# Autodesk Inventor assembly: Zahnriemen 16mm
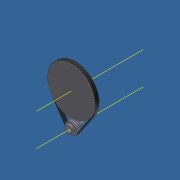
[picture p0: Inventor's stored thumbnail of the model, 180x180]
Saved by Autodesk Inventor 2016 (Build 200138000, 138)
## iProperties
Created: 2015-01-06
Document SubType Name: Assembly
Designer: 4ndreas
Mass: 1893.12 g
Surface Area: 594.287 cm^2
Volume: 258.329 cm^3
Density: 7.32831 g/cm^3
Part Number: Zahnriemen 16mm
ClientObjectVersion: 1
Author: 4ndreas
Title: 16mm Riemen
## Documents named in this file (4)
- C:\Users\4ndreas\Documents\Inventor\RobotARM v2\v2\BaseJoint\Konstruktions-Assistent\Übertragung des Zahnriemens1.iam
- C:\Users\4ndreas\Documents\Inventor\RobotARM v2\v2\BaseJoint\Konstruktions-Assistent\Zahnriemen1.ipt
- C:\Users\4ndreas\Documents\Inventor\RobotARM v2\v2\BaseJoint\Konstruktions-Assistent\Synchrone Riemenscheibe11.ipt
- C:\Users\4ndreas\Documents\Inventor\RobotARM v2\v2\BaseJoint\Konstruktions-Assistent\Synchrone Riemenscheibe21.ipt
## Components (3 placed, 3 different names)
1. Zahnriemen:1 — Fluchtend:1, Passend:1, Passend:2, Fluchtend:2, Passend:3, Passend:4
2. Synchrone Riemenscheibe1:1 — Fluchtend:1, Passend:1, Passend:2, Drehung:1
3. Synchrone Riemenscheibe2:1 — Fluchtend:2, Passend:3, Drehung:1, Passend:4
## Relationships (7: Mate 4, Flush 2, RelateRotation 1)
- Fluchtend:1 [Flush]: Zahnriemen:1 ↔ Synchrone Riemenscheibe1:1
- Passend:1 [Mate]: Zahnriemen:1 ↔ Synchrone Riemenscheibe1:1
- Passend:2 [Mate]: Zahnriemen:1 ↔ Synchrone Riemenscheibe1:1
- Fluchtend:2 [Flush]: Zahnriemen:1 ↔ Synchrone Riemenscheibe2:1
- Passend:3 [Mate]: Zahnriemen:1 ↔ Synchrone Riemenscheibe2:1
- Drehung:1 [RelateRotation] (0.1951 ul): Synchrone Riemenscheibe1:1 ↔ Synchrone Riemenscheibe2:1
- Passend:4 [Mate]: Zahnriemen:1 ↔ Synchrone Riemenscheibe2:1
